# Autodesk Inventor assembly: FullAssem
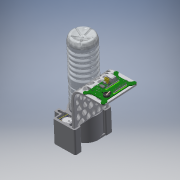
[picture p0: Inventor's stored thumbnail of the model, 180x180]
Saved by Autodesk Inventor 2019 (Build 230136000, 136)
## iProperties
Created: 2019-04-09
Part Number: FullAssem
Document SubType Name: Assembly
Designer: Jorian Brusind
Author: Jorian Brusind
## Documents named in this file (6)
- C:\Users\Jorian Brusind\Documents\GitHub\PersonalProjects\Automated Terrarium Project\Inventor Files\V3\FullAssem.iam
- C:\Users\Jorian Brusind\Documents\GitHub\PersonalProjects\Automated Terrarium Project\Inventor Files\V3\mini_pump.ipt
- C:\Users\Jorian Brusind\Documents\GitHub\PersonalProjects\Automated Terrarium Project\Inventor Files\V3\Bottle 600ml.iam
- C:\Users\Jorian Brusind\Documents\GitHub\PersonalProjects\Automated Terrarium Project\Inventor Files\V3\BoitCase.ipt
- C:\Users\Jorian Brusind\Documents\GitHub\PersonalProjects\Automated Terrarium Project\Inventor Files\V3\Backplate v1.ipt
- C:\Users\Jorian Brusind\Documents\GitHub\PersonalProjects\Automated Terrarium Project\Inventor Files\V3\AutoTerrarium.iam
## Components (5 placed, 5 different names)
1. Bottle 600ml:1 [sub-assembly] — Mate:2
2. BoitCase:1 — Mate:2, Mate:7, Mate:8, Mate:9, Mate:10
3. mini_pump:1 — Mate:7
4. Backplate v1:1 — Mate:8, Mate:9, Mate:10, Mate:11, Mate:12
5. AutoTerrarium:1 [sub-assembly] — Mate:11, Mate:12
## Relationships (7: Mate 7)
- Mate:2: Bottle 600ml:1 ↔ BoitCase:1
- Mate:7: BoitCase:1 ↔ mini_pump:1
- Mate:8: BoitCase:1 ↔ Backplate v1:1
- Mate:9 (0.5 mm): BoitCase:1 ↔ Backplate v1:1
- Mate:10 (0.5 mm): BoitCase:1 ↔ Backplate v1:1
- Mate:11: Backplate v1:1 ↔ AutoTerrarium:1
- Mate:12: Backplate v1:1 ↔ AutoTerrarium:1
